# Autodesk Inventor assembly: Wheel Hub
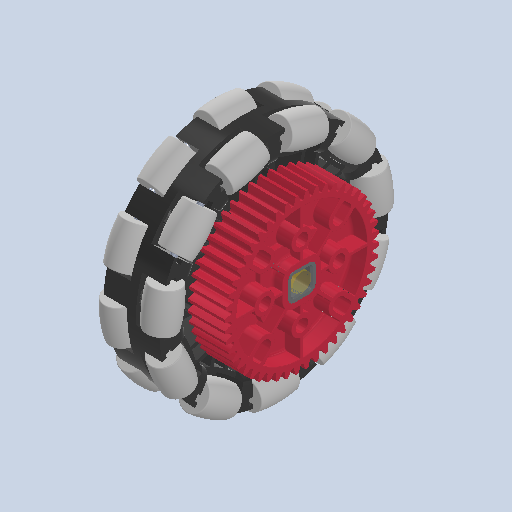
[picture p0: Inventor's stored thumbnail of the model, 512x512]
Saved by Autodesk Inventor 2025.2 (Build 292293000, 293)
## iProperties
Created: 2025-03-28
Part Number: Wheel Hub
Document SubType Name: Assembly
Designer: avere
Author: avere
## Documents named in this file (3)
- D:\vex\cad\v5\Drivetrain\Drivebay Right\Wheel Hub.iam
- D:\vex\cad\v5\Drivetrain\Drivebay Right\HS 48T Gear, No Insert.iam
- D:\vex\cad\v5\Drivetrain\Drivebay Right\3.25 Omni AS, No Insert.iam
## Components (2 placed, 2 different names)
1. HS 48T Gear, No Insert:1 [sub-assembly] — Insert:1
2. 3.25 Omni AS, No Insert:1 [sub-assembly] — Insert:1
## Relationships (1: Insert 1)
- Insert:1: HS 48T Gear, No Insert:1 ↔ 3.25 Omni AS, No Insert:1
